# Autodesk Inventor assembly: Adapter_drehteller
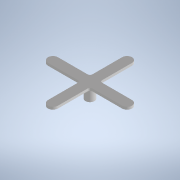
[picture p0: Inventor's stored thumbnail of the model, 180x180]
Saved by Autodesk Inventor 2021 (Build 250183000, 183)
## iProperties
Created: 2022-06-27
Part Number: Adapter_drehteller
Document SubType Name: Assembly
Designer: adria
Mass: 37.1629 g
Surface Area: 183.537 cm^2
Volume: 37.1629 cm^3
Density: 1 g/cm^3
Author: adria
## Documents named in this file (3)
- C:\Users\adria\OneDrive - tum.de\G2_Waste-Recycling\CAD\Adapter_drehteller.iam
- C:\Users\adria\OneDrive - tum.de\G2_Waste-Recycling\CAD\Adapter_Drehteller.ipt
- C:\Users\adria\OneDrive - tum.de\G2_Waste-Recycling\CAD\Clutch_nema.ipt
## Components (2 placed, 2 different names)
1. Adapter_Drehteller:1 — Passend:1, Passend:2
2. Clutch_nema:2 — Passend:1, Passend:2
## Relationships (2: Mate 2)
- Passend:1 [Mate]: Adapter_Drehteller:1 ↔ Clutch_nema:2
- Passend:2 [Mate]: Adapter_Drehteller:1 ↔ Clutch_nema:2
